# Autodesk Inventor assembly: CJ2D10-40Z(0_0)
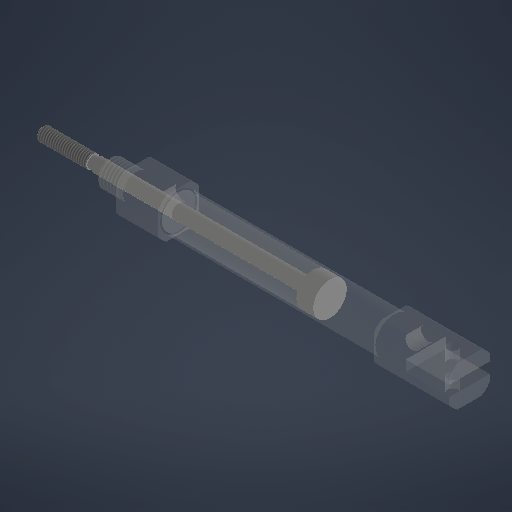
[picture p0: Inventor's stored thumbnail of the model, 512x512]
Saved by Autodesk Inventor 2025.2 (Build 292293000, 293)
## iProperties
Category: PARTsolutions
Company: SMC
Created: 2025-12-04
Part Number: CJ2D10-40Z(0_0)
Catalog Web Link: www.3dfindit.com
Description: CJ2-Z/CDJ2-Z-Air Cylinder/Standard: Double Acting Single Rod
Vendor: SMC
Document SubType Name: Assembly
Designer: psAdmin
Manufacturer: SMC
Mass: 8.42093 g
Surface Area: 83.0884 cm^2
Volume: 8.42093 cm^3
Density: 1 g/cm^3
PSOL_IDENT_0: {$CADENAS_DATA/23d-libs/smc_jp/actuator/standard_air_cylinder/cj2/cj2_z_asmtab.prj},300 {VTYP=3D},{S
PSOL_IDENT_1: TYP=ASSTAB},{NB=CJ2D10-40Z(0_0)},{LINA=CJ2D10-40Z},{NN=CJ2-Z/CDJ2-Z},{DATE=21.08.2025 09:02:40},{GEO
PSOL_IDENT_2: MDATE=08.08.2025 00:20:55},{VERSION=},{LINEID=390},{WBVAR=MAGNET,AUTOSWITCH,LEAD,NUMBER,CUSHION,STRO
PSOL_IDENT_3: KE,POS,PORT,BRACKET,RODB,MOUNTING,OMSC,OMSCXC3,OMSCXC51,THREAD},{WBNUMERIC=STROKE,POS}  {NB=CJ2D10-4
PSOL_IDENT_4: 0Z(0_0)},{LINA=CJ2D10-40Z},{KT=DUMMY},{NENN=CJ2D10-40Z},{ORDER=CJ2D10-40Z},{BORE=10},{MOUNT=(D) Doub
PSOL_IDENT_5: le clevis},{MOUNTX=D},{MAGNET=},{AUTOSWITCH=},{AUTOSWX='','N/A'},{LEAD=},{LEADX= '','N/A' },{NUMBER=
PSOL_IDENT_6: },{CUSHION=},{CUSHIONX= '','(-) Rubber cushion','A','(A) Air cushion' },{SWSIGNX= '','N/A' },{STROKE=
PSOL_IDENT_7: 40},{COM=Please confirm the conditions of use with SMC},{STDSTROKE=15,30,45,60,75,100,125,150},{STRO
PSOL_IDENT_8: KE1X=<20>,[2:400/1]},{SMIN=2},{SMINASW1=10},{SMINASW2=15},{SMAX1=400},{POS=0},{PORT=},{COM1=-},{BRAC
PSOL_IDENT_9: KET=},{RODB=},{RODBX= '', '(-) None', 'V', '(V) Single knuckle joint', 'W'  , '(W) Double knuckle jo
PSOL_IDENT_10: int', 'T', '(T) Rod end cap (Flat type)', 'U'  , '(U) Rod end cap (Round type)' },{MOUNTING=},{OMSC=
PSOL_IDENT_11: },{OMSCXC3=},{OMSCXC51=},{THREAD=0},{MOUNTINGX='','N/A'},{BRACKETX='','(-) None','N','(N) Pivot brac
PSOL_IDENT_12: ket is shipped together with the product,but not assembled.'},{PORTX='', '(-) Perpendicular to axis'
PSOL_IDENT_13: },{SW=B},{OMSCX= '','(-) None','-XB6','(XB6) Heat resistant cylinder (-10 to 150 degree Celsius)','-
PSOL_IDENT_14: XB7','(XB7) Cold resistant cylinder (-40 to 70 degree Celsius)','-XB9','(XB9) Low speed cylinder (10
PSOL_IDENT_15: to 50 mm/s)','-XC22','(XC22) Fluororubber seals','-XC85','(XC85) Grease specification for food proc
PSOL_IDENT_16: essing machines', '-X446'  , '(X446) PTFE grease' },{A=2.5},{XC3= '','(-) None','-XC3AB','(XC3AB) Ro
PSOL_IDENT_17: d port location viewed: A,Head port location viewed: B','-XC3AC','(XC3AC) Rod port location viewed:
PSOL_IDENT_18: A,Head port location viewed: C','-XC3AD','(XC3AD) Rod port location viewed: A,Head port location vie
PSOL_IDENT_19: wed: D','-XC3BA','(XC3BA) Rod port location viewed: B,Head port location viewed: A','-XC3BB','(XC3BB
PSOL_IDENT_20: ) Rod port location viewed: B,Head port location viewed: B','-XC3BC','(XC3BC) Rod port location view
PSOL_IDENT_21: ed: B,Head port location viewed: C','-XC3BD','(XC3BD) Rod port location viewed: B,Head port location
PSOL_IDENT_22: viewed: D','-XC3CA','(XC3CA) Rod port location viewed: C,Head port location viewed: A','-XC3CB','(X
PSOL_IDENT_23: C3CB) Rod port location viewed: C,Head port location viewed: B','-XC3CC','(XC3CC) Rod port location
PSOL_IDENT_24: viewed: C,Head port location viewed: C','-XC3CD','(XC3CD) Rod port location viewed: C,Head port loca
PSOL_IDENT_25: tion viewed: D','-XC3DA','(XC3DA) Rod port location viewed: D,Head port location viewed: A','-XC3DB'
PSOL_IDENT_26: ,'(XC3DB) Rod port location viewed: D,Head port location viewed: B','-XC3DC','(XC3DC) Rod port locat
PSOL_IDENT_27: ion viewed: D,Head port location viewed: C','-XC3DD','(XC3DD) Rod port location viewed: D,Head port
PSOL_IDENT_28: location viewed: D' },{XC51= '','(-) None','-XC51H4','(XC51H4) Hose nipple type: ø4/2.5 with restric
PSOL_IDENT_29: tion','-XC51H6','(XC51H6) Hose nipple type: ø6/4 with restriction','-XC51MH4','(XC51MH4) Hose nipple
PSOL_IDENT_30: type: ø4/2.5 without restriction','-XC51MH6','(XC51MH6) Hose nipple type: ø6/4 without restriction'
PSOL_IDENT_31: },{BMP=D},{PPATH=cj2_z/assembly/cj2_z_asmsbl.prj},{OMSCXX= '','(-) None','-XB6','(XB6) Heat resista
PSOL_IDENT_32: nt cylinder (-10 to 150 degree Celsius)','-XB7','(XB7) Cold resistant cylinder (-40 to 70 degree Cel
PSOL_IDENT_33: sius)','-XB9','(XB9) Low speed cylinder (10 to 50 mm/s)','-XC22','(XC22) Fluororubber seals','-XC85'
PSOL_IDENT_34: ,'(XC85) Grease specification for food processing machines', '-X446' , '(X446) PTFE grease' ,'-X2838'
PSOL_IDENT_35: ,'(X2838) Double clevis (With one-touch connecting pin)' }
NB: CJ2D10-40Z(0_0)
NN: CJ2-Z/CDJ2-Z
NT: Air Cylinder/Standard: Double Acting Single Rod
NBSYN: $ORDER.($POS._$THREAD.)
LINA: CJ2D10-40Z
CATALOG: SMC (JP
BORE: 10
MOUNT: (D) Double clevis
MAGNET: (-) Without magnet
AUTOSWITCH: N/A
LEAD: N/A
NUMBER: N/A
CUSHION: (-) Rubber cushion
STROKE: 40
POS: 0
PORT: (-) Perpendicular to axis
COM1: -
BRACKET: (-) None
RODB: (-) None
MOUNTING: N/A
OMSC: (-) None
OMSCXC3: (-) None
OMSCXC51: (-) None
THREAD: on
SUPPLIER: SMC
ARTICLENO: CJ2D10-40Z(0_0)
BOMINFO: CJ2D10-40Z
CREATOR: CADENAS GmbH
Title: CJ2D10-40Z
Author: Cadenas PARTsolutions
Comments: Air Cylinder/Standard: Double Acting Single Rod
## Documents named in this file (3)
- C:\Users\cloudy\Documents\GitHub\aura-cad\15\40 stroke 10 bore piston\CJ2D10-40Z(0_0).iam
- C:\Users\cloudy\Documents\GitHub\aura-cad\15\40 stroke 10 bore piston\CJ2D10-40Z(1_0)_BODY.ipt
- C:\Users\cloudy\Documents\GitHub\aura-cad\15\40 stroke 10 bore piston\CJ2D10-40Z_ROD.ipt
## Components (2 placed, 2 different names)
1. CJ2D10-40Z(1_0)_BODY:1 — Insert:1
2. CJ2D10-40Z_ROD:1 — Insert:1
## Relationships (1: Insert 1)
- Insert:1: CJ2D10-40Z(1_0)_BODY:1 ↔ CJ2D10-40Z_ROD:1
